# Autodesk Inventor assembly: SAR330  x 5 front + limit switches
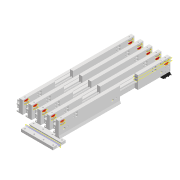
[picture p0: Inventor's stored thumbnail of the model, 180x180]
Saved by Autodesk Inventor 2020 (Build 240168000, 168)
## iProperties
Created: 2019-11-17
Part Number: SAR330  x 5 front + limit switches
Document SubType Name: Assembly
Designer: ball
Author: ball
## Documents named in this file (4)
- C:\FTC\FTC8863CAD\2019 Robot\Delivery\SAR330  x 5 front + limit switches.iam
- C:\FTC\FTC8863CAD\2019 Robot\Delivery\SAR330  x 5 + front couplers.iam
- C:\FTC\FTC8863CAD\Actobotics\605 parts\605630.ipt
- C:\FTC\FTC8863CAD\2019 Robot\Delivery\Coupler receiver.ipt
## Components (3 placed, 3 different names)
1. SAR330  x 5 + front couplers:1 [sub-assembly] — Flush:1, Flush:2, Mate:1, Mate:2
2. 605630:1 — Flush:1, Flush:2, Mate:1
3. Coupler receiver:1 — Mate:2
## Relationships (4: Flush 2, Mate 2)
- Flush:1: SAR330  x 5 + front couplers:1 ↔ 605630:1
- Flush:2: SAR330  x 5 + front couplers:1 ↔ 605630:1
- Mate:1 (2.54 mm): SAR330  x 5 + front couplers:1 ↔ 605630:1
- Mate:2 (25.4 mm): SAR330  x 5 + front couplers:1 ↔ Coupler receiver:1
